# Autodesk Inventor assembly: Assy_fork_left_test
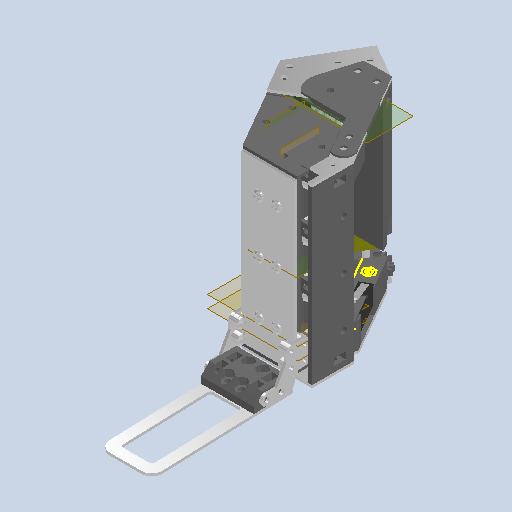
[picture p0: Inventor's stored thumbnail of the model, 512x512]
Saved by Autodesk Inventor 2024.1 (Build 281209000, 209)
## iProperties
Created: 2025-01-17
Part Number: Assy_fork_left_test
Document SubType Name: Assembly
Designer: hibik
Author: hibik
## Documents named in this file (5)
- C:\Users\hibik\Documents\Robomech\RESCUE\ORCA\hard\fork\Assy_fork_left_test.iam
- C:\Users\hibik\Documents\Robomech\RESCUE\ORCA\hard\fork\right\base_wall_added_MIR.iam
- C:\Users\hibik\Documents\Robomech\RESCUE\ORCA\hard\fork\right\screw_MIR.iam
- C:\Users\hibik\Documents\Robomech\RESCUE\ORCA\hard\fork\right\rail_MIR.iam
- C:\Users\hibik\Documents\Robomech\RESCUE\ORCA\hard\fork\right\motor_set_MIR.iam
## Components (4 placed, 4 different names)
1. base_wall_added_MIR:1 [sub-assembly] — 挿入:1, 正接:4, 正接:3, 正接:2, 正接:1, 角度:1, 挿入:2
2. screw_MIR:1 [sub-assembly] — 挿入:1
3. rail_MIR:1 [sub-assembly] — 正接:4, 正接:3, 正接:2, 正接:1
4. motor_set_MIR:1 [sub-assembly] — 角度:1, 挿入:2
## Relationships (7: Tangent 4, Insert 2, Angle 1)
- 挿入:1 [Insert]: base_wall_added_MIR:1 ↔ screw_MIR:1
- 正接:4 [Tangent]: base_wall_added_MIR:1 ↔ rail_MIR:1
- 正接:3 [Tangent]: base_wall_added_MIR:1 ↔ rail_MIR:1
- 正接:2 [Tangent]: base_wall_added_MIR:1 ↔ rail_MIR:1
- 正接:1 [Tangent]: base_wall_added_MIR:1 ↔ rail_MIR:1
- 角度:1 [Angle] (0 deg): base_wall_added_MIR:1 ↔ motor_set_MIR:1
- 挿入:2 [Insert]: base_wall_added_MIR:1 ↔ motor_set_MIR:1
